# Autodesk Inventor assembly: main
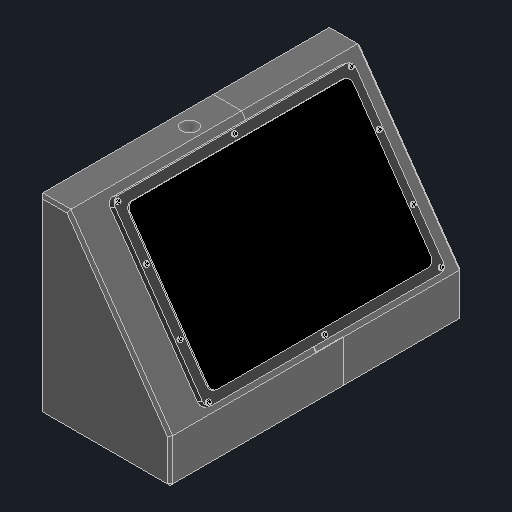
[picture p0: Inventor's stored thumbnail of the model, 512x512]
Saved by Autodesk Inventor 2026.2 (Build 302298000, 298)
## iProperties
Created: 2025-12-22
Part Number: main
Document SubType Name: Assembly
Designer: test
wood_thickness: 10.000 mm
Author: test
## Documents named in this file (12)
- D:\Projects\spl-monitor\simple-concert-monitor_Mechanical\main.iam
- D:\Projects\spl-monitor\simple-concert-monitor_Mechanical\external\raspberry-pi-4-model-b-1.snapshot.3\Raspberry Pi 4 Model B\Raspberry Pi 4 Model B\Raspberry Pi 4 Model B.iam
- D:\Projects\spl-monitor\simple-concert-monitor_Mechanical\external\adafruit-i2s-pi-mic-breakout-sph0645-1.snapshot.1\Pi Mic breakout SPH0645\Pi Mic breakout SPH0645\Pi Mic breakout SPH0645.ipt
- D:\Projects\spl-monitor\simple-concert-monitor_Mechanical\external\on-off-kcd4-220v-6a-1.snapshot.1\ON-OFF KCD4 220V 6A\ON-OFF KCD4 220V 6A\ON-OFF KCD4 220V 6A.iam
- D:\Projects\spl-monitor\simple-concert-monitor_Mechanical\external\ss-7b-as-207-ac-1-1.snapshot.3\SS-7B Socket\Plug SS-7B\Plug SS-7B\Plug SS-7B.ipt
- D:\Projects\spl-monitor\simple-concert-monitor_Mechanical\case3.ipt
- D:\Projects\spl-monitor\simple-concert-monitor_Mechanical\case4.ipt
- D:\Projects\spl-monitor\simple-concert-monitor_Mechanical\case5.ipt
- D:\Projects\spl-monitor\simple-concert-monitor_Mechanical\distances.ipt
- D:\Projects\spl-monitor\simple-concert-monitor_Mechanical\screen\pcb.ipt
- D:\Projects\spl-monitor\simple-concert-monitor_Mechanical\screen\screen_module.ipt
- D:\Projects\spl-monitor\simple-concert-monitor_Mechanical\screen\screw.ipt
## Components (23 placed, 11 different names)
1. Raspberry Pi 4 Model B:1 [sub-assembly] — Mate:21, Mate:22, Mate:23
2. Pi Mic breakout SPH0645:1 — Mate:24, Mate:25, Mate:26
3. ON-OFF KCD4 220V 6A:1 [sub-assembly] — Mate:6, Mate:7, Mate:8
4. Plug SS-7B:1 — Mate:5, Mate:9, Mate:10
5. case3:1 — Flush:1, Mate:12, Flush:2, Mate:13, Mate:14, Mate:15, Mate:16, Mate:17, Mate:18, Mate:19, Mate:20, Mate:24, Mate:25, Mate:26, Flush:3, Mate:27, Mate:28, Mate:31, Mate:32
6. case4:1 — Flush:1, Mate:5, Mate:6, Mate:7, Mate:8, Mate:9, Mate:10, Mate:11, Flush:3, Mate:29, Mate:30
7. case5:1 — Mate:11, Mate:12, Flush:2
8. distances:1 — Mate:13, Mate:14, Mate:21
9. distances:2 — Mate:15, Mate:16
10. distances:3 — Mate:17, Mate:18
11. distances:4 — Mate:19, Mate:20, Mate:22, Mate:23
12. pcb:1 — Mate:30, Mate:31, Mate:32
13. screen_module:1 — Mate:27, Mate:28, Mate:29, Rigid:1, Rotational:1, Rotational:2, Rotational:3, Rigid:2, Rigid:3, Rigid:4, Rotational:4, Rigid:5, Rigid:6
14. screw:1 — Rigid:6
15. screw:2 — Rigid:1
16. screw:3 — Rotational:1
17. screw:4 — Rotational:2
18. screw:5 — Rotational:3
19. screw:6 — Rigid:2
20. screw:7 — Rigid:3
21. screw:8 — Rigid:4
22. screw:9 — Rotational:4
23. screw:10 — Rigid:5
## Relationships (41: Mate 28, WeldJoint 6, RevoluteJoint 4, Flush 3)
- Flush:1: case3:1 ↔ case4:1
- Mate:5: Plug SS-7B:1 ↔ case4:1
- Mate:6: ON-OFF KCD4 220V 6A:1 ↔ case4:1
- Mate:7: ON-OFF KCD4 220V 6A:1 ↔ case4:1
- Mate:8: ON-OFF KCD4 220V 6A:1 ↔ case4:1
- Mate:9: Plug SS-7B:1 ↔ case4:1
- Mate:10: Plug SS-7B:1 ↔ case4:1
- Mate:11: case4:1 ↔ case5:1
- Mate:12: case3:1 ↔ case5:1
- Flush:2: case3:1 ↔ case5:1
- Mate:13: case3:1 ↔ distances:1
- Mate:14: case3:1 ↔ distances:1
- Mate:15: case3:1 ↔ distances:2
- Mate:16: case3:1 ↔ distances:2
- Mate:17: case3:1 ↔ distances:3
- Mate:18: case3:1 ↔ distances:3
- Mate:19: case3:1 ↔ distances:4
- Mate:20: case3:1 ↔ distances:4
- Mate:21: Raspberry Pi 4 Model B:1 ↔ distances:1
- Mate:22: Raspberry Pi 4 Model B:1 ↔ distances:4
- Mate:23: Raspberry Pi 4 Model B:1 ↔ distances:4
- Mate:24: Pi Mic breakout SPH0645:1 ↔ case3:1
- Mate:25: Pi Mic breakout SPH0645:1 ↔ case3:1
- Mate:26: Pi Mic breakout SPH0645:1 ↔ case3:1
- Flush:3: case3:1 ↔ case4:1
- Mate:27: case3:1 ↔ screen_module:1
- Mate:28: case3:1 ↔ screen_module:1
- Mate:29: case4:1 ↔ screen_module:1
- Mate:30: case4:1 ↔ pcb:1
- Mate:31: case3:1 ↔ pcb:1
- Mate:32: case3:1 ↔ pcb:1
- Rigid:1 [WeldJoint]: screen_module:1 ↔ screw:2
- Rotational:1 [RevoluteJoint]: screen_module:1 ↔ screw:3
- Rotational:2 [RevoluteJoint]: screen_module:1 ↔ screw:4
- Rotational:3 [RevoluteJoint]: screen_module:1 ↔ screw:5
- Rigid:2 [WeldJoint]: screen_module:1 ↔ screw:6
- Rigid:3 [WeldJoint]: screen_module:1 ↔ screw:7
- Rigid:4 [WeldJoint]: screen_module:1 ↔ screw:8
- Rotational:4 [RevoluteJoint]: screen_module:1 ↔ screw:9
- Rigid:5 [WeldJoint]: screen_module:1 ↔ screw:10
- Rigid:6 [WeldJoint]: screen_module:1 ↔ screw:1
